# Autodesk Inventor assembly: Assembly1
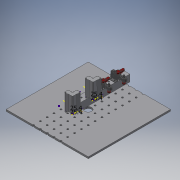
[picture p0: Inventor's stored thumbnail of the model, 180x180]
Saved by Autodesk Inventor 2018 (Build 220112000, 112)
## iProperties
Created: 2018-12-05
Part Number: Assembly1
Document SubType Name: Assembly
Designer: gbgic
Author: gbgic
## Documents named in this file (5)
- C:\Users\Gabriel\Documents\GitHub\2019CAD\Assembly1.iam
- C:\Users\Gabriel\Documents\GitHub\2019CAD\Drill Jig Base.ipt
- C:\Users\Gabriel\Documents\GitHub\2019CAD\Tube Beam.ipt
- C:\Users\Gabriel\Documents\GitHub\2019CAD\305-U.iam
- C:\Users\Gabriel\Documents\GitHub\2019CAD\Jig2.1_1x1_Bolt_Pattern_PIN.ipt
## Components (6 placed, 4 different names)
1. Drill Jig Base:1 — Mate:1, Mate:2, Mate:3
2. Tube Beam:1 — Mate:1, Mate:2, Mate:3, Angle:1, Mate:4, Mate:5, Mate:6
3. 305-U:1 [sub-assembly] — Angle:1, Mate:4
4. 305-U:2 [sub-assembly] — Mate:5, Mate:6
5. Jig2.1_1x1_Bolt_Pattern_PIN:1
6. Jig2.1_1x1_Bolt_Pattern_PIN:2
## Relationships (7: Mate 6, Angle 1)
- Mate:1: Drill Jig Base:1 ↔ Tube Beam:1
- Mate:2: Drill Jig Base:1 ↔ Tube Beam:1
- Mate:3: Drill Jig Base:1 ↔ Tube Beam:1
- Angle:1 (0 deg): Tube Beam:1 ↔ 305-U:1
- Mate:4: Tube Beam:1 ↔ 305-U:1
- Mate:5: Tube Beam:1 ↔ 305-U:2
- Mate:6: Tube Beam:1 ↔ 305-U:2
